# Autodesk Inventor assembly: PAL
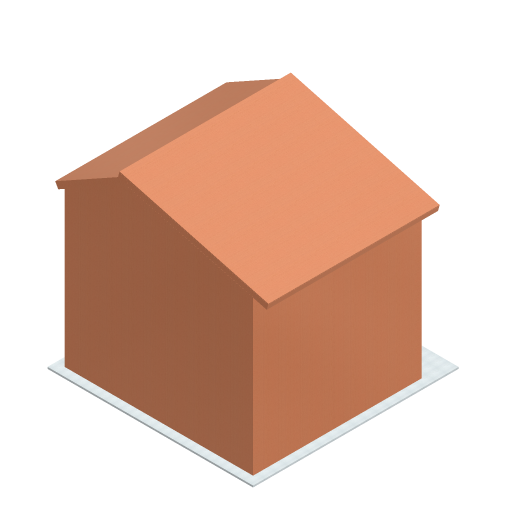
[picture p0: Inventor's stored thumbnail of the model, 512x512]
Saved by Autodesk Inventor 2024 (Build 280153000, 153)
## iProperties
Created: 2024-11-29
Part Number: PAL
Document SubType Name: Assembly
Designer: dasam
Author: dasam
## Documents named in this file (7)
- C:\Users\dasam\OneDrive - De Vinci\Innovation project & technological expedition\3D models\PAL V3\PAL.iam
- C:\Users\dasam\OneDrive - De Vinci\Innovation project & technological expedition\3D models\PAL V2\Back panel.ipt
- C:\Users\dasam\OneDrive - De Vinci\Innovation project & technological expedition\3D models\PAL V2\Floor.ipt
- C:\Users\dasam\OneDrive - De Vinci\Innovation project & technological expedition\3D models\PAL V2\Front panel.ipt
- C:\Users\dasam\OneDrive - De Vinci\Innovation project & technological expedition\3D models\PAL V2\Large ceiling.ipt
- C:\Users\dasam\OneDrive - De Vinci\Innovation project & technological expedition\3D models\PAL V2\Short ceiling.ipt
- C:\Users\dasam\OneDrive - De Vinci\Innovation project & technological expedition\3D models\PAL V2\Side panel.ipt
## Components (7 placed, 6 different names)
1. Back panel:1 — Mate:5, Mate:8, Flush:5, Flush:6, Mate:9, Mate:10, Flush:7, Flush:8
2. Floor:1 — Mate:1, Mate:2, Mate:5, Mate:6, Flush:4, Flush:6
3. Front panel:1 — Mate:1, Mate:3, Mate:7, Flush:1, Flush:2, Mate:11
4. Large ceiling:1 — Mate:9, Mate:10, Flush:7, Mate:12
5. Short ceiling:1 — Mate:11, Mate:12, Flush:8
6. Side panel:1 — Mate:6, Mate:7, Flush:2, Flush:5
7. Side panel:2 — Mate:2, Mate:3, Flush:1, Flush:4, Mate:8
## Relationships (18: Mate 11, Flush 7)
- Mate:1: Floor:1 ↔ Front panel:1
- Mate:2: Floor:1 ↔ Side panel:2
- Mate:3: Front panel:1 ↔ Side panel:2
- Mate:5: Back panel:1 ↔ Floor:1
- Mate:6: Floor:1 ↔ Side panel:1
- Mate:7: Front panel:1 ↔ Side panel:1
- Flush:1: Front panel:1 ↔ Side panel:2
- Flush:2: Front panel:1 ↔ Side panel:1
- Flush:4 (100 mm): Floor:1 ↔ Side panel:2
- Mate:8: Back panel:1 ↔ Side panel:2
- Flush:5: Back panel:1 ↔ Side panel:1
- Flush:6 (100 mm): Back panel:1 ↔ Floor:1
- Mate:9: Back panel:1 ↔ Large ceiling:1
- Mate:10 (-100 mm): Back panel:1 ↔ Large ceiling:1
- Flush:7: Back panel:1 ↔ Large ceiling:1
- Mate:11: Front panel:1 ↔ Short ceiling:1
- Mate:12: Large ceiling:1 ↔ Short ceiling:1
- Flush:8: Back panel:1 ↔ Short ceiling:1
